# Autodesk Inventor assembly: _Design_TopOfLid
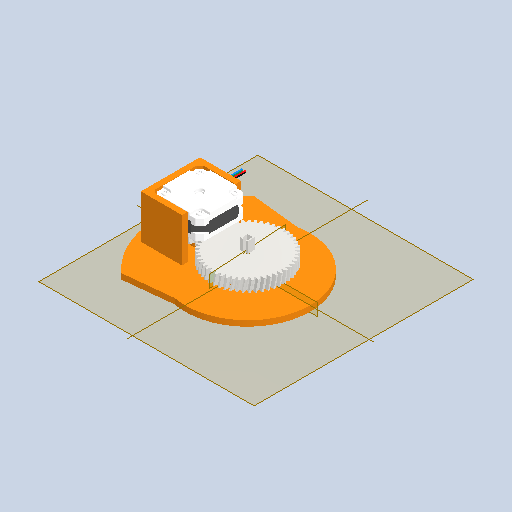
[picture p0: Inventor's stored thumbnail of the model, 512x512]
Saved by Autodesk Inventor 2023.2 (Build 272271030, 271C)
## iProperties
Created: 2023-06-04
Part Number: _Design_TopOfLid
Document SubType Name: Assembly
Designer: atrus
Author: atrus
## Documents named in this file (4)
- C:\Users\atrus\Dropbox\elec\Mechanical\SkimmerSwabbie\_Design_TopOfLid.iam
- C:\Users\atrus\Dropbox\elec\Mechanical\SkimmerSwabbie\TopGearPlate.ipt
- C:\Users\atrus\Dropbox\elec\Mechanical\SkimmerSwabbie\_GearTrain.iam
- C:\Users\atrus\Dropbox\elec\Mechanical\SkimmerSwabbie\17HS08-1004S\17HS08-1004S.ipt
## Components (3 placed, 3 different names)
1. TopGearPlate:1 — Mate:1, Mate:2, Angle:1, Mate:3, Tangent:1
2. _GearTrain:1 [sub-assembly] — Mate:1, Mate:2, Angle:1
3. 17HS08-1004S:1 — Mate:3, Tangent:1
## Relationships (5: Mate 3, Angle 1, Tangent 1)
- Mate:1: TopGearPlate:1 ↔ _GearTrain:1
- Mate:2: TopGearPlate:1 ↔ _GearTrain:1
- Angle:1 (180 deg): TopGearPlate:1 ↔ _GearTrain:1
- Mate:3: TopGearPlate:1 ↔ 17HS08-1004S:1
- Tangent:1: TopGearPlate:1 ↔ 17HS08-1004S:1
